# Autodesk Inventor assembly: Assembly1
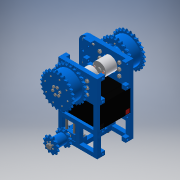
[picture p0: Inventor's stored thumbnail of the model, 180x180]
Saved by Autodesk Inventor 2016 (Build 200138000, 138)
## iProperties
Created: 2016-06-04
Part Number: Assembly1
Document SubType Name: Assembly
Designer: hesaon
Author: hesaon
## Documents named in this file (27)
- C:\Users\hesaon\Documents\Killer-Bot-2016\AutodeskWorkspace\robotparts revision 2\Assembly1.iam
- C:\Users\hesaon\Documents\Killer-Bot-2016\AutodeskWorkspace\robotparts revision 2\sideFrame.ipt
- C:\Users\hesaon\Documents\Killer-Bot-2016\AutodeskWorkspace\robotparts revision 2\motorHolder57mmVer2.ipt
- C:\Users\hesaon\Documents\Killer-Bot-2016\AutodeskWorkspace\robotparts revision 2\nut4mm.ipt
- C:\Users\hesaon\Documents\Killer-Bot-2016\AutodeskWorkspace\robotparts revision 2\screw18x4mm.ipt
- C:\Users\hesaon\Documents\Killer-Bot-2016\AutodeskWorkspace\robotparts revision 2\washer4mm.ipt
- C:\Users\hesaon\Documents\Killer-Bot-2016\AutodeskWorkspace\robotparts revision 2\37D mm metal gearmotor.ipt
- C:\Users\hesaon\Documents\Killer-Bot-2016\AutodeskWorkspace\robotparts revision 2\washer3mm.ipt
- C:\Users\hesaon\Documents\Killer-Bot-2016\AutodeskWorkspace\robotparts revision 2\screw12x3mm.ipt
- C:\Users\hesaon\Documents\Killer-Bot-2016\AutodeskWorkspace\robotparts revision 2\mountingHub6mm.ipt
- C:\Users\hesaon\Documents\Killer-Bot-2016\AutodeskWorkspace\robotparts revision 2\bigOuterSprocket.ipt
- C:\Users\hesaon\Documents\Killer-Bot-2016\AutodeskWorkspace\robotparts revision 2\bigSprocketsHolder.ipt
- C:\Users\hesaon\Documents\Killer-Bot-2016\AutodeskWorkspace\robotparts revision 2\bigInnerSprocket.ipt
- C:\Users\hesaon\Documents\Killer-Bot-2016\AutodeskWorkspace\robotparts revision 2\screwKa22x16.ipt
- C:\Users\hesaon\Documents\Killer-Bot-2016\AutodeskWorkspace\robotparts revision 2\battery.ipt
- C:\Users\hesaon\Documents\Killer-Bot-2016\AutodeskWorkspace\robotparts revision 2\backFrame.ipt
- C:\Users\hesaon\Documents\Killer-Bot-2016\AutodeskWorkspace\robotparts revision 2\screw27x4mm.ipt
- C:\Users\hesaon\Documents\Killer-Bot-2016\AutodeskWorkspace\robotparts revision 2\pin5x60.ipt
- C:\Users\hesaon\Documents\Killer-Bot-2016\AutodeskWorkspace\robotparts revision 2\smallSprocketFixture.ipt
- C:\Users\hesaon\Documents\Killer-Bot-2016\AutodeskWorkspace\robotparts revision 2\nut6mm.ipt
- C:\Users\hesaon\Documents\Killer-Bot-2016\AutodeskWorkspace\robotparts revision 2\washer6mm.ipt
- C:\Users\hesaon\Documents\Killer-Bot-2016\AutodeskWorkspace\robotparts revision 2\smallSprocketDistance.ipt
- C:\Users\hesaon\Documents\Killer-Bot-2016\AutodeskWorkspace\robotparts revision 2\smallSprocket.ipt
- C:\Users\hesaon\Documents\Killer-Bot-2016\AutodeskWorkspace\robotparts revision 2\smallSprocketHolder.ipt
- C:\Users\hesaon\Documents\Killer-Bot-2016\AutodeskWorkspace\robotparts revision 2\bolt90x6mm.ipt
- C:\Users\hesaon\Documents\Killer-Bot-2016\AutodeskWorkspace\robotparts revision 2\sideFrame2.ipt
- C:\Users\hesaon\Documents\Killer-Bot-2016\AutodeskWorkspace\robotparts revision 2\bottomSideFrame.ipt
## Components (231 placed, 25 different names)
1. sideFrame:1 — Insert:1, Insert:2, Insert:3, Insert:4, Insert:5, Insert:6, Insert:7, Insert:8, Mate:2, Insert:80, Insert:81, Insert:86, Insert:87, Insert:90, Insert:91, Insert:247, Insert:248, Insert:249, Insert:250
2. motorHolder57mmVer2:1 — Insert:1, Insert:2, Insert:9, Insert:10, Insert:11, Insert:12, Insert:13, Insert:14, Insert:27, Insert:28, Insert:29, Insert:30, Insert:31, Insert:32, Insert:33, Insert:34
3. nut4mm:1 — Insert:26
4. nut4mm:2 — Insert:21
5. nut4mm:3 — Insert:22
6. nut4mm:4 — Insert:23
7. nut4mm:5 — Insert:24
8. nut4mm:6 — Insert:25
9. screw18x4mm:1 — Insert:17
10. screw18x4mm:2 — Insert:19
11. screw18x4mm:3 — Insert:16
12. screw18x4mm:4 — Insert:15
13. screw18x4mm:5 — Insert:18
14. screw18x4mm:6 — Insert:20
15. washer4mm:1 — Insert:5, Insert:21
16. washer4mm:2 — Insert:8, Insert:24
17. washer4mm:3 — Insert:10, Insert:17
18. washer4mm:4 — Insert:9, Insert:15
19. washer4mm:5 — Insert:11, Insert:18
20. washer4mm:6 — Insert:12, Insert:19
21. washer4mm:7 — Insert:7, Insert:26
22. washer4mm:8 — Insert:13, Insert:16
23. washer4mm:9 — Insert:14, Insert:20
24. washer4mm:10 — Insert:4, Insert:23
25. washer4mm:11 — Insert:3, Insert:22
26. washer4mm:12 — Insert:6, Insert:25
27. 37D mm metal gearmotor:1 — Insert:27, Insert:28, Insert:41
28. washer3mm:1 — Insert:29, Insert:37
29. washer3mm:2 — Insert:30, Insert:36
30. washer3mm:3 — Insert:32, Insert:40
31. washer3mm:4 — Insert:31, Insert:35
32. washer3mm:5 — Insert:33, Insert:39
33. washer3mm:6 — Insert:34, Insert:38
34. screw12x3mm:1 — Insert:38
35. screw12x3mm:2 — Insert:35
36. screw12x3mm:3 — Insert:36
37. screw12x3mm:4 — Insert:37
38. screw12x3mm:5 — Insert:40
39. screw12x3mm:6 — Insert:39
40. mountingHub6mm:1 — Insert:41, Insert:42, Insert:43
41. Outer big sprocket:1 — Insert:42, Insert:43, Insert:44, Insert:45, Insert:48, Insert:49, Insert:50, Insert:51, Insert:52, Insert:53, Insert:54, Insert:55, Insert:64, Insert:65, Insert:66, Insert:67, Insert:68, Insert:69
42. bigSprocketsHolder:1 — Insert:44, Insert:45, Insert:46, Insert:47
43. Roller Chain Sprocket1:1 — Insert:46, Insert:47, Insert:56, Insert:57, Insert:58, Insert:59, Insert:60, Insert:61, Insert:62, Insert:63
44. screwKa22x16:1 — Insert:56
45. screwKa22x16:2 — Insert:57
46. screwKa22x16:3 — Insert:58
47. screwKa22x16:4 — Insert:59
48. screwKa22x16:5 — Insert:60
49. screwKa22x16:6 — Insert:61
50. screwKa22x16:7 — Insert:63
51. screwKa22x16:8 — Insert:62
52. screwKa22x16:9 — Insert:48
53. screwKa22x16:10 — Insert:49
54. screwKa22x16:11 — Insert:50
55. screwKa22x16:12 — Insert:51
56. screwKa22x16:13 — Insert:52
57. screwKa22x16:14 — Insert:53
58. screwKa22x16:15 — Insert:54
59. screwKa22x16:16 — Insert:55
60. washer3mm:7 — Insert:64, Insert:70
61. washer3mm:8 — Insert:65, Insert:74
62. washer3mm:9 — Insert:66, Insert:75
63. washer3mm:10 — Insert:67, Insert:73
64. washer3mm:11 — Insert:68, Insert:72
65. washer3mm:12 — Insert:69, Insert:71
66. screw12x3mm:7 — Insert:70
67. screw12x3mm:8 — Insert:71
68. screw12x3mm:9 — Insert:72
69. screw12x3mm:10 — Insert:73
70. screw12x3mm:11 — Insert:74
71. screw12x3mm:12 — Insert:75
72. battery:1 — Mate:2, Mate:4, Mate:5
73. backFrame:1 — Insert:86, Insert:87, Insert:88, Insert:89, Insert:117, Insert:118, Insert:119, Insert:120, Insert:121, Insert:122
74. nut4mm:7 — Insert:85
75. nut4mm:8 — Insert:84
76. washer4mm:13 — Insert:82, Insert:89
77. washer4mm:14 — Insert:83, Insert:88
78. washer4mm:15 — Insert:80, Insert:85
79. washer4mm:16 — Insert:81, Insert:84
80. screw27x4mm:1 — Insert:83
81. screw27x4mm:2 — Insert:82
82. pin5x60:1 — Insert:91, Cylindrical:2
83. pin5x60:2 — Insert:90, Cylindrical:1
84. smallSprocketFixture:1 — Cylindrical:1, Cylindrical:2, Insert:92, Angle:1, Insert:94
85. nut6mm:1 — Insert:92, Angle:1, Insert:93
86. washer6mm:1 — Insert:93, Insert:95
87. washer6mm:2 — Insert:94, Insert:116
88. smallSprocketDistance:1 — Insert:95, Insert:96
89. washer6mm:3 — Insert:96, Insert:97
90. Roller Chain Sprocket1:2 — Insert:100, Insert:101, Insert:102, Insert:103, Insert:104, Insert:105, Insert:106, Insert:107, Insert:114
91. Roller Chain Sprocket1:3 — Insert:97, Insert:98, Insert:99, Insert:108, Insert:109, Insert:110, Insert:111, Insert:112, Insert:113
92. smallSprocketHolder:1 — Insert:98, Insert:99, Insert:100, Insert:101
93. screwKa22x16:17 — Insert:111
94. screwKa22x16:18 — Insert:104
95. screwKa22x16:19 — Insert:105
96. screwKa22x16:20 — Insert:106
97. screwKa22x16:21 — Insert:107
98. screwKa22x16:22 — Insert:109
99. screwKa22x16:23 — Insert:110
100. screwKa22x16:24 — Insert:112
101. screwKa22x16:25 — Insert:113
102. screwKa22x16:26 — Insert:108
103. screwKa22x16:27 — Insert:103
104. screwKa22x16:28 — Insert:102
105. washer6mm:4 — Insert:114, Insert:115
106. bolt90x6mm:1 — Insert:115
107. nut6mm:2 — Insert:116
108. sideFrame2:1 — Insert:117, Insert:118, Insert:127, Insert:128, Insert:153, Insert:154, Insert:175, Insert:176, Insert:177, Insert:178, Insert:179, Insert:180, Insert:193, Insert:194, Insert:294, Insert:295, Insert:296, Mate:5
109. screw27x4mm:3 — Insert:125
110. screw27x4mm:4 — Insert:126
111. nut4mm:9 — Insert:124
112. nut4mm:10 — Insert:123
113. washer4mm:17 — Insert:122, Insert:124
114. washer4mm:18 — Insert:121, Insert:123
115. washer4mm:19 — Insert:120, Insert:125
116. washer4mm:20 — Insert:119, Insert:126
117. pin5x60:3 — Insert:128, Cylindrical:4
118. pin5x60:4 — Insert:127, Cylindrical:3
119. smallSprocketFixture:2 — Cylindrical:3, Cylindrical:4, Insert:129, Angle:2, Insert:130
120. nut6mm:3 — Insert:140
121. nut6mm:4 — Insert:129, Angle:2, Insert:131
122. washer6mm:5 — Insert:130, Insert:140
123. washer6mm:6 — Insert:131, Insert:132
124. washer6mm:7 — Insert:133, Insert:134
125. washer6mm:8 — Insert:138, Insert:139
126. smallSprocketDistance:2 — Insert:132, Insert:133
127. Roller Chain Sprocket1:4 — Insert:134, Insert:135, Insert:136, Insert:147, Insert:148, Insert:149, Insert:150, Insert:151, Insert:152
128. Roller Chain Sprocket1:5 — Insert:137, Mate:3, Insert:138, Insert:141, Insert:142, Insert:143, Insert:144, Insert:145, Insert:146
129. smallSprocketHolder:2 — Insert:135, Insert:136, Insert:137, Mate:3
130. bolt90x6mm:2 — Insert:139
131. screwKa22x16:29 — Insert:149
132. screwKa22x16:30 — Insert:150
133. screwKa22x16:31 — Insert:148
134. screwKa22x16:32 — Insert:151
135. screwKa22x16:33 — Insert:147
136. screwKa22x16:34 — Insert:152
137. screwKa22x16:35 — Insert:146
138. screwKa22x16:36 — Insert:143
139. screwKa22x16:37 — Insert:144
140. screwKa22x16:38 — Insert:145
141. screwKa22x16:39 — Insert:141
142. screwKa22x16:40 — Insert:142
143. motorHolder57mmVer2:2 — Insert:153, Insert:154, Insert:155, Insert:156, Insert:157, Insert:158, Insert:159, Insert:160, Insert:161, Insert:162, Insert:169, Insert:170, Insert:171, Insert:172, Insert:173, Insert:174
144. 37D mm metal gearmotor:2 — Insert:155, Insert:156, Insert:197
145. washer3mm:13 — Insert:157, Insert:168
146. washer3mm:14 — Insert:158, Insert:163
147. washer3mm:15 — Insert:159, Insert:164
148. washer3mm:16 — Insert:160, Insert:165
149. washer3mm:17 — Insert:161, Insert:166
150. washer3mm:18 — Insert:162, Insert:167
151. screw12x3mm:13 — Insert:163
152. screw12x3mm:14 — Insert:164
153. screw12x3mm:15 — Insert:165
154. screw12x3mm:16 — Insert:166
155. screw12x3mm:17 — Insert:167
156. screw12x3mm:18 — Insert:168
157. washer4mm:21 — Insert:169, Insert:181
158. washer4mm:22 — Insert:170, Insert:182
159. washer4mm:23 — Insert:172, Insert:184
160. washer4mm:24 — Insert:174, Insert:186
161. washer4mm:25 — Insert:173, Insert:185
162. washer4mm:26 — Insert:171, Insert:183
163. washer4mm:27 — Insert:180, Insert:189
164. washer4mm:28 — Insert:177, Insert:191
165. washer4mm:29 — Insert:178, Insert:188
166. washer4mm:30 — Insert:176, Insert:187
167. washer4mm:31 — Insert:179, Insert:192
168. washer4mm:32 — Insert:175, Insert:190
169. nut4mm:11 — Insert:188
170. nut4mm:12 — Insert:189
171. nut4mm:13 — Insert:191
172. nut4mm:14 — Insert:192
173. nut4mm:15 — Insert:190
174. nut4mm:16 — Insert:187
175. screw18x4mm:7 — Insert:183
176. screw18x4mm:8 — Insert:184
177. screw18x4mm:9 — Insert:185
178. screw18x4mm:10 — Insert:186
179. screw18x4mm:11 — Insert:182
180. screw18x4mm:12 — Insert:181
181. washer4mm:33 — Insert:193, Insert:195
182. washer4mm:34 — Insert:194, Insert:196
183. nut4mm:17 — Insert:195
184. nut4mm:18 — Insert:196
185. mountingHub6mm:2 — Insert:197, Insert:198, Insert:199, Insert:200
186. Outer big sprocket:2 — Insert:198, Insert:199, Insert:200, Insert:201, Insert:202, Insert:203, Insert:204, Insert:205, Insert:206, Insert:213, Insert:214, Insert:217, Insert:218, Insert:219, Insert:220, Insert:221, Insert:222, Insert:223, Insert:224
187. washer3mm:19 — Insert:202, Insert:211
188. washer3mm:20 — Insert:201, Insert:212
189. washer3mm:21 — Insert:203, Insert:210
190. washer3mm:22 — Insert:205, Insert:208
191. washer3mm:23 — Insert:204, Insert:209
192. washer3mm:24 — Insert:206, Insert:207
193. screw12x3mm:19 — Insert:207
194. screw12x3mm:20 — Insert:208
195. screw12x3mm:21 — Insert:209
196. screw12x3mm:22 — Insert:210
197. screw12x3mm:23 — Insert:211
198. screw12x3mm:24 — Insert:212
199. bigSprocketsHolder:2 — Insert:213, Insert:214, Insert:215, Insert:216
200. Roller Chain Sprocket1:6 — Insert:215, Insert:216, Insert:225, Insert:226, Insert:227, Insert:228, Insert:229, Insert:230, Insert:231, Insert:232
201. screwKa22x16:41 — Insert:232
202. screwKa22x16:42 — Insert:228
203. screwKa22x16:43 — Insert:226
204. screwKa22x16:44 — Insert:225
205. screwKa22x16:45 — Insert:224
206. screwKa22x16:46 — Insert:223
207. screwKa22x16:47 — Insert:222
208. screwKa22x16:48 — Insert:221
209. screwKa22x16:49 — Insert:220
210. screwKa22x16:50 — Insert:227
211. screwKa22x16:51 — Insert:231
212. screwKa22x16:52 — Insert:229
213. screwKa22x16:53 — Insert:230
214. screwKa22x16:54 — Insert:219
215. screwKa22x16:55 — Insert:218
216. screwKa22x16:56 — Insert:217
217. bottomSideFrame:1 — Insert:243, Insert:244, Insert:246, Insert:294, Insert:295, Insert:296, Mate:4
218. washer4mm:35 — Insert:243, Insert:251
219. washer4mm:36 — Insert:244, Insert:252
220. washer4mm:38 — Insert:246, Insert:253
221. washer4mm:39 — Insert:247, Insert:255
222. washer4mm:40 — Insert:248, Insert:256
223. washer4mm:41 — Insert:250, Insert:258
224. washer4mm:42 — Insert:249, Insert:257
225. screw27x4mm:5 — Insert:251
226. screw27x4mm:6 — Insert:252
227. screw27x4mm:7 — Insert:253
228. nut4mm:19 — Insert:255
229. nut4mm:20 — Insert:256
230. nut4mm:21 — Insert:258
231. nut4mm:22 — Insert:257
## Relationships (255: Insert 245, Mate 4, CylindricalJoint 4, Angle 2)
- Insert:1: sideFrame:1 ↔ motorHolder57mmVer2:1
- Insert:2: sideFrame:1 ↔ motorHolder57mmVer2:1
- Insert:3: sideFrame:1 ↔ washer4mm:11
- Insert:4: sideFrame:1 ↔ washer4mm:10
- Insert:5: sideFrame:1 ↔ washer4mm:1
- Insert:6: sideFrame:1 ↔ washer4mm:12
- Insert:7: sideFrame:1 ↔ washer4mm:7
- Insert:8: sideFrame:1 ↔ washer4mm:2
- Insert:9: motorHolder57mmVer2:1 ↔ washer4mm:4
- Insert:10: motorHolder57mmVer2:1 ↔ washer4mm:3
- Insert:11: motorHolder57mmVer2:1 ↔ washer4mm:5
- Insert:12: motorHolder57mmVer2:1 ↔ washer4mm:6
- Insert:13: motorHolder57mmVer2:1 ↔ washer4mm:8
- Insert:14: motorHolder57mmVer2:1 ↔ washer4mm:9
- Insert:15: screw18x4mm:4 ↔ washer4mm:4
- Insert:16: screw18x4mm:3 ↔ washer4mm:8
- Insert:17: screw18x4mm:1 ↔ washer4mm:3
- Insert:18: screw18x4mm:5 ↔ washer4mm:5
- Insert:19: screw18x4mm:2 ↔ washer4mm:6
- Insert:20: screw18x4mm:6 ↔ washer4mm:9
- Insert:21: nut4mm:2 ↔ washer4mm:1
- Insert:22: nut4mm:3 ↔ washer4mm:11
- Insert:23: nut4mm:4 ↔ washer4mm:10
- Insert:24: nut4mm:5 ↔ washer4mm:2
- Insert:25: nut4mm:6 ↔ washer4mm:12
- Insert:26: nut4mm:1 ↔ washer4mm:7
- Insert:27: motorHolder57mmVer2:1 ↔ 37D mm metal gearmotor:1
- Insert:28: motorHolder57mmVer2:1 ↔ 37D mm metal gearmotor:1
- Insert:29: motorHolder57mmVer2:1 ↔ washer3mm:1
- Insert:30: motorHolder57mmVer2:1 ↔ washer3mm:2
- Insert:31: motorHolder57mmVer2:1 ↔ washer3mm:4
- Insert:32: motorHolder57mmVer2:1 ↔ washer3mm:3
- Insert:33: motorHolder57mmVer2:1 ↔ washer3mm:5
- Insert:34: motorHolder57mmVer2:1 ↔ washer3mm:6
- Insert:35: washer3mm:4 ↔ screw12x3mm:2
- Insert:36: washer3mm:2 ↔ screw12x3mm:3
- Insert:37: washer3mm:1 ↔ screw12x3mm:4
- Insert:38: washer3mm:6 ↔ screw12x3mm:1
- Insert:39: washer3mm:5 ↔ screw12x3mm:6
- Insert:40: washer3mm:3 ↔ screw12x3mm:5
- Insert:41: 37D mm metal gearmotor:1 ↔ mountingHub6mm:1
- Insert:42: mountingHub6mm:1 ↔ Outer big sprocket:1
- Insert:43: mountingHub6mm:1 ↔ Outer big sprocket:1
- Insert:44: Outer big sprocket:1 ↔ bigSprocketsHolder:1
- Insert:45: Outer big sprocket:1 ↔ bigSprocketsHolder:1
- Insert:46: bigSprocketsHolder:1 ↔ Roller Chain Sprocket1:1
- Insert:47: bigSprocketsHolder:1 ↔ Roller Chain Sprocket1:1
- Insert:48: Outer big sprocket:1 ↔ screwKa22x16:9
- Insert:49: Outer big sprocket:1 ↔ screwKa22x16:10
- Insert:50: Outer big sprocket:1 ↔ screwKa22x16:11
- Insert:51: Outer big sprocket:1 ↔ screwKa22x16:12
- Insert:52: Outer big sprocket:1 ↔ screwKa22x16:13
- Insert:53: Outer big sprocket:1 ↔ screwKa22x16:14
- Insert:54: Outer big sprocket:1 ↔ screwKa22x16:15
- Insert:55: Outer big sprocket:1 ↔ screwKa22x16:16
- Insert:56: Roller Chain Sprocket1:1 ↔ screwKa22x16:1
- Insert:57: Roller Chain Sprocket1:1 ↔ screwKa22x16:2
- Insert:58: Roller Chain Sprocket1:1 ↔ screwKa22x16:3
- Insert:59: Roller Chain Sprocket1:1 ↔ screwKa22x16:4
- Insert:60: Roller Chain Sprocket1:1 ↔ screwKa22x16:5
- Insert:61: Roller Chain Sprocket1:1 ↔ screwKa22x16:6
- Insert:62: Roller Chain Sprocket1:1 ↔ screwKa22x16:8
- Insert:63: Roller Chain Sprocket1:1 ↔ screwKa22x16:7
- Insert:64: Outer big sprocket:1 ↔ washer3mm:7
- Insert:65: Outer big sprocket:1 ↔ washer3mm:8
- Insert:66: Outer big sprocket:1 ↔ washer3mm:9
- Insert:67: Outer big sprocket:1 ↔ washer3mm:10
- Insert:68: Outer big sprocket:1 ↔ washer3mm:11
- Insert:69: Outer big sprocket:1 ↔ washer3mm:12
- Insert:70: washer3mm:7 ↔ screw12x3mm:7
- Insert:71: washer3mm:12 ↔ screw12x3mm:8
- Insert:72: washer3mm:11 ↔ screw12x3mm:9
- Insert:73: washer3mm:10 ↔ screw12x3mm:10
- Insert:74: washer3mm:8 ↔ screw12x3mm:11
- Insert:75: washer3mm:9 ↔ screw12x3mm:12
- Mate:2: sideFrame:1 ↔ battery:1
- Insert:80: sideFrame:1 ↔ washer4mm:15
- Insert:81: sideFrame:1 ↔ washer4mm:16
- Insert:82: washer4mm:13 ↔ screw27x4mm:2
- Insert:83: washer4mm:14 ↔ screw27x4mm:1
- Insert:84: nut4mm:8 ↔ washer4mm:16
- Insert:85: nut4mm:7 ↔ washer4mm:15
- Insert:86: sideFrame:1 ↔ backFrame:1
- Insert:87: sideFrame:1 ↔ backFrame:1
- Insert:88: backFrame:1 ↔ washer4mm:14
- Insert:89: backFrame:1 ↔ washer4mm:13
- Insert:90: sideFrame:1 ↔ pin5x60:2
- Insert:91: sideFrame:1 ↔ pin5x60:1
- Cylindrical:1: pin5x60:2 ↔ smallSprocketFixture:1
- Cylindrical:2: pin5x60:1 ↔ smallSprocketFixture:1
- Insert:92: smallSprocketFixture:1 ↔ nut6mm:1
- Angle:1 (0 deg): smallSprocketFixture:1 ↔ nut6mm:1
- Insert:93: nut6mm:1 ↔ washer6mm:1
- Insert:94: smallSprocketFixture:1 ↔ washer6mm:2
- Insert:95: washer6mm:1 ↔ smallSprocketDistance:1
- Insert:96: smallSprocketDistance:1 ↔ washer6mm:3
- Insert:97: washer6mm:3 ↔ Roller Chain Sprocket1:3
- Insert:98: Roller Chain Sprocket1:3 ↔ smallSprocketHolder:1
- Insert:99: Roller Chain Sprocket1:3 ↔ smallSprocketHolder:1
- Insert:100: Roller Chain Sprocket1:2 ↔ smallSprocketHolder:1
- Insert:101: Roller Chain Sprocket1:2 ↔ smallSprocketHolder:1
- Insert:102: Roller Chain Sprocket1:2 ↔ screwKa22x16:28
- Insert:103: Roller Chain Sprocket1:2 ↔ screwKa22x16:27
- Insert:104: Roller Chain Sprocket1:2 ↔ screwKa22x16:18
- Insert:105: Roller Chain Sprocket1:2 ↔ screwKa22x16:19
- Insert:106: Roller Chain Sprocket1:2 ↔ screwKa22x16:20
- Insert:107: Roller Chain Sprocket1:2 ↔ screwKa22x16:21
- Insert:108: Roller Chain Sprocket1:3 ↔ screwKa22x16:26
- Insert:109: Roller Chain Sprocket1:3 ↔ screwKa22x16:22
- Insert:110: Roller Chain Sprocket1:3 ↔ screwKa22x16:23
- Insert:111: Roller Chain Sprocket1:3 ↔ screwKa22x16:17
- Insert:112: Roller Chain Sprocket1:3 ↔ screwKa22x16:24
- Insert:113: Roller Chain Sprocket1:3 ↔ screwKa22x16:25
- Insert:114: Roller Chain Sprocket1:2 ↔ washer6mm:4
- Insert:115: washer6mm:4 ↔ bolt90x6mm:1
- Insert:116: washer6mm:2 ↔ nut6mm:2
- Insert:117: backFrame:1 ↔ sideFrame2:1
- Insert:118: backFrame:1 ↔ sideFrame2:1
- Insert:119: backFrame:1 ↔ washer4mm:20
- Insert:120: backFrame:1 ↔ washer4mm:19
- Insert:121: backFrame:1 ↔ washer4mm:18
- Insert:122: backFrame:1 ↔ washer4mm:17
- Insert:123: nut4mm:10 ↔ washer4mm:18
- Insert:124: nut4mm:9 ↔ washer4mm:17
- Insert:125: screw27x4mm:3 ↔ washer4mm:19
- Insert:126: screw27x4mm:4 ↔ washer4mm:20
- Insert:127: sideFrame2:1 ↔ pin5x60:4
- Insert:128: sideFrame2:1 ↔ pin5x60:3
- Cylindrical:3: pin5x60:4 ↔ smallSprocketFixture:2
- Cylindrical:4: pin5x60:3 ↔ smallSprocketFixture:2
- Insert:129: smallSprocketFixture:2 ↔ nut6mm:4
- Angle:2 (0 deg): smallSprocketFixture:2 ↔ nut6mm:4
- Insert:130: smallSprocketFixture:2 ↔ washer6mm:5
- Insert:131: nut6mm:4 ↔ washer6mm:6
- Insert:132: washer6mm:6 ↔ smallSprocketDistance:2
- Insert:133: washer6mm:7 ↔ smallSprocketDistance:2
- Insert:134: washer6mm:7 ↔ Roller Chain Sprocket1:4
- Insert:135: Roller Chain Sprocket1:4 ↔ smallSprocketHolder:2
- Insert:136: Roller Chain Sprocket1:4 ↔ smallSprocketHolder:2
- Insert:137: Roller Chain Sprocket1:5 ↔ smallSprocketHolder:2
- Mate:3: Roller Chain Sprocket1:5 ↔ smallSprocketHolder:2
- Insert:138: washer6mm:8 ↔ Roller Chain Sprocket1:5
- Insert:139: washer6mm:8 ↔ bolt90x6mm:2
- Insert:140: nut6mm:3 ↔ washer6mm:5
- Insert:141: Roller Chain Sprocket1:5 ↔ screwKa22x16:39
- Insert:142: Roller Chain Sprocket1:5 ↔ screwKa22x16:40
- Insert:143: Roller Chain Sprocket1:5 ↔ screwKa22x16:36
- Insert:144: Roller Chain Sprocket1:5 ↔ screwKa22x16:37
- Insert:145: Roller Chain Sprocket1:5 ↔ screwKa22x16:38
- Insert:146: Roller Chain Sprocket1:5 ↔ screwKa22x16:35
- Insert:147: Roller Chain Sprocket1:4 ↔ screwKa22x16:33
- Insert:148: Roller Chain Sprocket1:4 ↔ screwKa22x16:31
- Insert:149: Roller Chain Sprocket1:4 ↔ screwKa22x16:29
- Insert:150: Roller Chain Sprocket1:4 ↔ screwKa22x16:30
- Insert:151: Roller Chain Sprocket1:4 ↔ screwKa22x16:32
- Insert:152: Roller Chain Sprocket1:4 ↔ screwKa22x16:34
- Insert:153: sideFrame2:1 ↔ motorHolder57mmVer2:2
- Insert:154: sideFrame2:1 ↔ motorHolder57mmVer2:2
- Insert:155: motorHolder57mmVer2:2 ↔ 37D mm metal gearmotor:2
- Insert:156: motorHolder57mmVer2:2 ↔ 37D mm metal gearmotor:2
- Insert:157: motorHolder57mmVer2:2 ↔ washer3mm:13
- Insert:158: motorHolder57mmVer2:2 ↔ washer3mm:14
- Insert:159: motorHolder57mmVer2:2 ↔ washer3mm:15
- Insert:160: motorHolder57mmVer2:2 ↔ washer3mm:16
- Insert:161: motorHolder57mmVer2:2 ↔ washer3mm:17
- Insert:162: motorHolder57mmVer2:2 ↔ washer3mm:18
- Insert:163: washer3mm:14 ↔ screw12x3mm:13
- Insert:164: washer3mm:15 ↔ screw12x3mm:14
- Insert:165: washer3mm:16 ↔ screw12x3mm:15
- Insert:166: washer3mm:17 ↔ screw12x3mm:16
- Insert:167: washer3mm:18 ↔ screw12x3mm:17
- Insert:168: washer3mm:13 ↔ screw12x3mm:18
- Insert:169: motorHolder57mmVer2:2 ↔ washer4mm:21
- Insert:170: motorHolder57mmVer2:2 ↔ washer4mm:22
- Insert:171: motorHolder57mmVer2:2 ↔ washer4mm:26
- Insert:172: motorHolder57mmVer2:2 ↔ washer4mm:23
- Insert:173: motorHolder57mmVer2:2 ↔ washer4mm:25
- Insert:174: motorHolder57mmVer2:2 ↔ washer4mm:24
- Insert:175: sideFrame2:1 ↔ washer4mm:32
- Insert:176: sideFrame2:1 ↔ washer4mm:30
- Insert:177: sideFrame2:1 ↔ washer4mm:28
- Insert:178: sideFrame2:1 ↔ washer4mm:29
- Insert:179: sideFrame2:1 ↔ washer4mm:31
- Insert:180: sideFrame2:1 ↔ washer4mm:27
- Insert:181: washer4mm:21 ↔ screw18x4mm:12
- Insert:182: washer4mm:22 ↔ screw18x4mm:11
- Insert:183: washer4mm:26 ↔ screw18x4mm:7
- Insert:184: washer4mm:23 ↔ screw18x4mm:8
- Insert:185: washer4mm:25 ↔ screw18x4mm:9
- Insert:186: washer4mm:24 ↔ screw18x4mm:10
- Insert:187: washer4mm:30 ↔ nut4mm:16
- Insert:188: washer4mm:29 ↔ nut4mm:11
- Insert:189: washer4mm:27 ↔ nut4mm:12
- Insert:190: washer4mm:32 ↔ nut4mm:15
- Insert:191: washer4mm:28 ↔ nut4mm:13
- Insert:192: washer4mm:31 ↔ nut4mm:14
- Insert:193: sideFrame2:1 ↔ washer4mm:33
- Insert:194: sideFrame2:1 ↔ washer4mm:34
- Insert:195: washer4mm:33 ↔ nut4mm:17
- Insert:196: washer4mm:34 ↔ nut4mm:18
- Insert:197: 37D mm metal gearmotor:2 ↔ mountingHub6mm:2
- Insert:198: mountingHub6mm:2 ↔ Outer big sprocket:2
- Insert:199: mountingHub6mm:2 ↔ Outer big sprocket:2
- Insert:200: mountingHub6mm:2 ↔ Outer big sprocket:2
- Insert:201: Outer big sprocket:2 ↔ washer3mm:20
- Insert:202: Outer big sprocket:2 ↔ washer3mm:19
- Insert:203: Outer big sprocket:2 ↔ washer3mm:21
- Insert:204: Outer big sprocket:2 ↔ washer3mm:23
- Insert:205: Outer big sprocket:2 ↔ washer3mm:22
- Insert:206: Outer big sprocket:2 ↔ washer3mm:24
- Insert:207: washer3mm:24 ↔ screw12x3mm:19
- Insert:208: washer3mm:22 ↔ screw12x3mm:20
- Insert:209: washer3mm:23 ↔ screw12x3mm:21
- Insert:210: washer3mm:21 ↔ screw12x3mm:22
- Insert:211: washer3mm:19 ↔ screw12x3mm:23
- Insert:212: washer3mm:20 ↔ screw12x3mm:24
- Insert:213: Outer big sprocket:2 ↔ bigSprocketsHolder:2
- Insert:214: Outer big sprocket:2 ↔ bigSprocketsHolder:2
- Insert:215: bigSprocketsHolder:2 ↔ Roller Chain Sprocket1:6
- Insert:216: bigSprocketsHolder:2 ↔ Roller Chain Sprocket1:6
- Insert:217: Outer big sprocket:2 ↔ screwKa22x16:56
- Insert:218: Outer big sprocket:2 ↔ screwKa22x16:55
- Insert:219: Outer big sprocket:2 ↔ screwKa22x16:54
- Insert:220: Outer big sprocket:2 ↔ screwKa22x16:49
- Insert:221: Outer big sprocket:2 ↔ screwKa22x16:48
- Insert:222: Outer big sprocket:2 ↔ screwKa22x16:47
- Insert:223: Outer big sprocket:2 ↔ screwKa22x16:46
- Insert:224: Outer big sprocket:2 ↔ screwKa22x16:45
- Insert:225: Roller Chain Sprocket1:6 ↔ screwKa22x16:44
- Insert:226: Roller Chain Sprocket1:6 ↔ screwKa22x16:43
- Insert:227: Roller Chain Sprocket1:6 ↔ screwKa22x16:50
- Insert:228: Roller Chain Sprocket1:6 ↔ screwKa22x16:42
- Insert:229: Roller Chain Sprocket1:6 ↔ screwKa22x16:52
- Insert:230: Roller Chain Sprocket1:6 ↔ screwKa22x16:53
- Insert:231: Roller Chain Sprocket1:6 ↔ screwKa22x16:51
- Insert:232: Roller Chain Sprocket1:6 ↔ screwKa22x16:41
- Insert:243: bottomSideFrame:1 ↔ washer4mm:35
- Insert:244: bottomSideFrame:1 ↔ washer4mm:36
- Insert:246: bottomSideFrame:1 ↔ washer4mm:38
- Insert:247: sideFrame:1 ↔ washer4mm:39
- Insert:248: sideFrame:1 ↔ washer4mm:40
- Insert:249: sideFrame:1 ↔ washer4mm:42
- Insert:250: sideFrame:1 ↔ washer4mm:41
- Insert:251: washer4mm:35 ↔ screw27x4mm:5
- Insert:252: washer4mm:36 ↔ screw27x4mm:6
- Insert:253: washer4mm:38 ↔ screw27x4mm:7
- Insert:255: washer4mm:39 ↔ nut4mm:19
- Insert:256: washer4mm:40 ↔ nut4mm:20
- Insert:257: washer4mm:42 ↔ nut4mm:22
- Insert:258: washer4mm:41 ↔ nut4mm:21
- Insert:294: sideFrame2:1 ↔ bottomSideFrame:1
- Insert:295: sideFrame2:1 ↔ bottomSideFrame:1
- Insert:296: sideFrame2:1 ↔ bottomSideFrame:1
- Mate:4: battery:1 ↔ bottomSideFrame:1
- Mate:5: battery:1 ↔ sideFrame2:1
